# Autodesk Inventor assembly: RCR_ArmAssemblyFinal
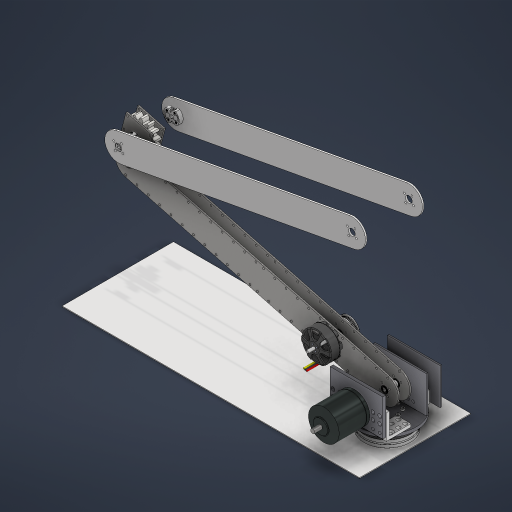
[picture p0: Inventor's stored thumbnail of the model, 512x512]
Saved by Autodesk Inventor 2024 (Build 280153000, 153)
## iProperties
Created: 2023-11-20
Part Number: RCR_ArmAssemblyFinal
Document SubType Name: Assembly
Designer: avsar
Author: avsar
## Documents named in this file (24)
- C:\Users\avsar\Documents\Inventor\RCR_Arm_Temp\ArmFinal\RCR_ArmAssemblyFinal.iam
- C:\Users\avsar\Documents\Inventor\RCR_Arm_Temp\Chassis\ChassisTop V3.ipt
- C:\Users\avsar\Documents\Inventor\RCR_Arm_Temp\COTS\Motion\Bearings\Crossed Roller Bearings\35mm Shaft Crossed Roller Bearing.ipt
- C:\Users\avsar\Documents\Inventor\RCR_Arm_Temp\ArmFinal\Turret\TurretPulley.ipt
- C:\Users\avsar\Documents\Inventor\RCR_Arm_Temp\ArmFinal\Turret\TurretBasePlate.ipt
- C:\Users\avsar\Documents\Inventor\RCR_Arm_Temp\COTS\ISO Standard Hardware\Screws\Sockethead Screws\Cap Screws\M4 x 0.7mm\(M4 x 0.7 x 30) Sockethead Cap Screw.ipt
- C:\Users\avsar\Documents\Inventor\RCR_Arm_Temp\COTS\Motion\Actuation\Motors\BLDC Motors\ODrive BLDC Motor - D6374 150KV.ipt
- C:\Users\avsar\Documents\Inventor\RCR_Arm_Temp\COTS\Motion\Actuation\Motors\BLDC Motors\ODrive Dual Shaft Motor - D5312s 330KV.ipt
- C:\Users\avsar\Documents\Inventor\RCR_Arm_Temp\ArmFinal\ArmStages\FirstStageMotorPlate.ipt
- C:\Users\avsar\Documents\Inventor\RCR_Arm_Temp\ArmFinal\ArmStages\ArmSupportPlate.ipt
- C:\Users\avsar\Documents\Inventor\RCR_Arm_Temp\ArmFinal\ArmStages\FirstStageArmBar1.ipt
- C:\Users\avsar\Documents\Inventor\RCR_Arm_Temp\COTS\goBilda\Motion\Bearings\(8mm REX ID x 14mm OD, 5mm Thickness) 1611 Series Flanged Ball Bearing.ipt
- C:\Users\avsar\Documents\Inventor\RCR_Arm_Temp\ArmFinal\ArmStages\ArmPlateSpacerFirstStage.ipt
- C:\Users\avsar\Documents\Inventor\RCR_Arm_Temp\COTS\goBilda\Motion\Collars\8mm REX-Shaft Set Screw Collar.ipt
- C:\Users\avsar\Documents\Inventor\RCR_Arm_Temp\ArmFinal\ArmStages\FirstArmStageSupportSpacer.ipt
- C:\Users\avsar\Documents\Inventor\RCR_Arm_Temp\COTS\ISO Standard Hardware\Screws\Sockethead Screws\Cap Screws\M4 x 0.7mm\(M4 x 0.7 x 8) Sockethead Cap Screw.ipt
- C:\Users\avsar\Documents\Inventor\RCR_Arm_Temp\ArmFinal\ArmStages\LongL-Bracket.ipt
- C:\Users\avsar\Documents\Inventor\RCR_Arm_Temp\ArmFinal\ArmStages\SecondArmStageMotorPulley.ipt
- C:\Users\avsar\Documents\Inventor\RCR_Arm_Temp\COTS\goBilda\Motion\Hubs\Sonic Hubs\Sonic Hub (8mm REX Bore).ipt
- C:\Users\avsar\Documents\Inventor\RCR_Arm_Temp\COTS\goBilda\Motion\Axles\(8mm Diameter, 56mm Length) 2106 Series Threaded REX Shaft with E-Clip.ipt
- C:\Users\avsar\Documents\Inventor\RCR_Arm_Temp\COTS\goBilda\Motion\Collars\Clamping Collar (8mm Rex).ipt
- C:\Users\avsar\Documents\Inventor\RCR_Arm_Temp\ArmFinal\ArmStages\SecondStageGears\ArmGears_SecondStage\Design Accelerator\Spur Gear11.ipt
- C:\Users\avsar\Documents\Inventor\RCR_Arm_Temp\ArmFinal\ArmStages\SecondStageArmBar.ipt
- C:\Users\avsar\Documents\Inventor\RCR_Arm_Temp\ArmFinal\ArmStages\ArmSupport_C-Channel.ipt
## Components (49 placed, 23 different names)
1. ChassisTop V3:1 — Mate:1, Mate:2, Mate:3
2. 35mm Shaft Crossed Roller Bearing:1 — Mate:1, Mate:2, Mate:3, Mate:4, Mate:5
3. TurretPulley:1 — Mate:4, Mate:5, Mate:6, Mate:7, Mate:8
4. (M4 x 0.7 x 30) Sockethead Cap Screw:1 — Mate:13, Mate:14
5. (M4 x 0.7 x 30) Sockethead Cap Screw:2 — Mate:11, Mate:12
6. (M4 x 0.7 x 30) Sockethead Cap Screw:3 — Mate:9, Mate:10
7. (M4 x 0.7 x 30) Sockethead Cap Screw:4 — Mate:19, Mate:20
8. (M4 x 0.7 x 30) Sockethead Cap Screw:5 — Mate:17, Mate:18
9. (M4 x 0.7 x 30) Sockethead Cap Screw:6 — Mate:15, Mate:16
10. TurretBasePlate:1 — Mate:6, Mate:7, Mate:8, Mate:9, Mate:10, Mate:11, Mate:12, Mate:13, Mate:14, Mate:15, Mate:16, Mate:17, Mate:18, Mate:19, Mate:20, Mate:21, Mate:22, Mate:23, Mate:24, Mate:77, Mate:80, Mate:119, Mate:120, Mate:121
11. (M4 x 0.7 x 30) Sockethead Cap Screw:7 — Mate:23, Mate:24
12. (M4 x 0.7 x 30) Sockethead Cap Screw:8 — Mate:21, Mate:22
13. ODrive Dual Shaft Motor - D5312s 330KV:1 — Mate:52, Mate:53, Mate:54
14. FirstStageMotorPlate:1 — Mate:36, Mate:37, Mate:38, Mate:70, Mate:71, Mate:74, Mate:75, Mate:76, Mate:78, Mate:79
15. ODrive BLDC Motor - D6374 150KV:3 — Mate:36, Mate:37, Mate:38, Mate:51
16. ArmSupportPlate:1 — Mate:123, Mate:126, Mate:127
17. ArmSupportPlate:2 — Mate:65, Mate:66, Mate:122, Mate:124, Mate:125
18. FirstStageArmBar1:1 — Mate:51, Mate:52, Mate:53, Mate:54, Mate:55, Flush:2, Mate:56, Mate:57, Mate:89, Mate:90, Mate:91, Mate:92, Mate:106
19. FirstStageArmBar1:2 — Mate:55, Flush:2, Mate:58, Mate:59, Mate:81, Mate:82, Mate:86, Mate:87, Mate:88, Mate:93, Mate:94
20. (8mm REX ID x 14mm OD, 5mm Thickness) 1611 Series Flanged Ball Bearing:1 — Mate:56, Mate:57, Mate:62
21. (8mm REX ID x 14mm OD, 5mm Thickness) 1611 Series Flanged Ball Bearing:2 — Mate:58, Mate:59, Mate:60, Mate:61, Mate:69
22. ArmPlateSpacerFirstStage:1 — Mate:60, Mate:61, Mate:63, Mate:64, Mate:68
23. 8mm REX-Shaft Set Screw Collar:1 — Mate:62, Mate:63, Mate:64
24. (8mm REX ID x 14mm OD, 5mm Thickness) 1611 Series Flanged Ball Bearing:3 — Mate:65, Mate:66, Mate:67, Mate:128
25. FirstArmStageSupportSpacer:1 — Mate:67, Mate:68, Mate:69, Mate:128
26. (M4 x 0.7 x 8) Sockethead Cap Screw:1 — Mate:70, Mate:71
27. (M4 x 0.7 x 8) Sockethead Cap Screw:2 — Mate:74, Mate:75
28. LongL-Bracket:1 — Mate:76, Mate:77, Mate:78, Mate:79, Mate:80
29. SecondArmStageMotorPulley:1 — Mate:81, Mate:82, Flush:3
30. SecondArmStageMotorPulley:2 — Mate:83, Mate:84, Mate:85, Flush:3, Mate:86, Mate:95, Mate:96
31. Sonic Hub (8mm REX Bore):1 — Mate:83, Mate:84, Mate:85
32. (8mm REX ID x 14mm OD, 5mm Thickness) 1611 Series Flanged Ball Bearing:4 — Mate:87, Mate:88
33. (8mm REX ID x 14mm OD, 5mm Thickness) 1611 Series Flanged Ball Bearing:5 — Mate:89, Mate:90, Mate:97, Mate:98
34. (8mm REX ID x 14mm OD, 5mm Thickness) 1611 Series Flanged Ball Bearing:6 — Mate:91, Mate:92, Mate:110, Mate:112, Mate:129, Mate:130
35. (8mm REX ID x 14mm OD, 5mm Thickness) 1611 Series Flanged Ball Bearing:7 — Mate:93, Mate:94, Mate:111, Mate:131, Mate:132
36. (8mm REX ID x 14mm OD, 5mm Thickness) 1611 Series Flanged Ball Bearing:8 — Mate:95, Mate:96, Mate:99
37. (8mm Diameter, 56mm Length) 2106 Series Threaded REX Shaft with E-Clip:1 — Mate:97, Mate:98, Mate:100, Mate:101, Mate:105
38. Clamping Collar (8mm Rex):1 — Mate:99, Mate:100, Mate:101
39. Spur Gear1:1 — Mate:102, Mate:103, Mate:104, Mate:105, Mate:106, Flush:4
40. Sonic Hub (8mm REX Bore):2 — Mate:102, Mate:103, Mate:104
41. Spur Gear1:2 — Mate:110, Flush:4
42. Sonic Hub (8mm REX Bore):3 — Flush:8
43. SecondStageArmBar:1 — Mate:111, Flush:5, Mate:113, Mate:114, Mate:115
44. SecondStageArmBar:2 — Mate:112, Flush:5, Mate:116, Mate:117, Mate:118
45. Sonic Hub (8mm REX Bore):4 — Mate:113, Mate:114, Mate:115, Flush:6, Flush:7, Flush:8
46. Sonic Hub (8mm REX Bore):5 — Mate:116, Mate:117, Mate:118, Mate:133
47. ArmSupport_C-Channel:1 — Mate:119, Mate:120, Mate:121, Mate:122, Mate:123, Mate:124, Mate:125, Mate:126, Mate:127
48. Clamping Collar (8mm Rex):2 — Mate:129, Mate:130, Flush:6
49. Clamping Collar (8mm Rex):3 — Mate:131, Mate:132, Flush:7, Mate:133
## Relationships (115: Mate 108, Flush 7)
- Mate:1: ChassisTop V3:1 ↔ 35mm Shaft Crossed Roller Bearing:1
- Mate:2: ChassisTop V3:1 ↔ 35mm Shaft Crossed Roller Bearing:1
- Mate:3: ChassisTop V3:1 ↔ 35mm Shaft Crossed Roller Bearing:1
- Mate:4: 35mm Shaft Crossed Roller Bearing:1 ↔ TurretPulley:1
- Mate:5: 35mm Shaft Crossed Roller Bearing:1 ↔ TurretPulley:1
- Mate:6: TurretPulley:1 ↔ TurretBasePlate:1
- Mate:7: TurretPulley:1 ↔ TurretBasePlate:1
- Mate:8: TurretPulley:1 ↔ TurretBasePlate:1
- Mate:9: (M4 x 0.7 x 30) Sockethead Cap Screw:3 ↔ TurretBasePlate:1
- Mate:10: (M4 x 0.7 x 30) Sockethead Cap Screw:3 ↔ TurretBasePlate:1
- Mate:11: (M4 x 0.7 x 30) Sockethead Cap Screw:2 ↔ TurretBasePlate:1
- Mate:12: (M4 x 0.7 x 30) Sockethead Cap Screw:2 ↔ TurretBasePlate:1
- Mate:13: (M4 x 0.7 x 30) Sockethead Cap Screw:1 ↔ TurretBasePlate:1
- Mate:14: (M4 x 0.7 x 30) Sockethead Cap Screw:1 ↔ TurretBasePlate:1
- Mate:15: (M4 x 0.7 x 30) Sockethead Cap Screw:6 ↔ TurretBasePlate:1
- Mate:16: (M4 x 0.7 x 30) Sockethead Cap Screw:6 ↔ TurretBasePlate:1
- Mate:17: (M4 x 0.7 x 30) Sockethead Cap Screw:5 ↔ TurretBasePlate:1
- Mate:18: (M4 x 0.7 x 30) Sockethead Cap Screw:5 ↔ TurretBasePlate:1
- Mate:19: (M4 x 0.7 x 30) Sockethead Cap Screw:4 ↔ TurretBasePlate:1
- Mate:20: (M4 x 0.7 x 30) Sockethead Cap Screw:4 ↔ TurretBasePlate:1
- Mate:21: TurretBasePlate:1 ↔ (M4 x 0.7 x 30) Sockethead Cap Screw:8
- Mate:22: TurretBasePlate:1 ↔ (M4 x 0.7 x 30) Sockethead Cap Screw:8
- Mate:23: TurretBasePlate:1 ↔ (M4 x 0.7 x 30) Sockethead Cap Screw:7
- Mate:24: TurretBasePlate:1 ↔ (M4 x 0.7 x 30) Sockethead Cap Screw:7
- Mate:36: FirstStageMotorPlate:1 ↔ ODrive BLDC Motor - D6374 150KV:3
- Mate:37: FirstStageMotorPlate:1 ↔ ODrive BLDC Motor - D6374 150KV:3
- Mate:38: FirstStageMotorPlate:1 ↔ ODrive BLDC Motor - D6374 150KV:3
- Mate:51: ODrive BLDC Motor - D6374 150KV:3 ↔ FirstStageArmBar1:1
- Mate:52: ODrive Dual Shaft Motor - D5312s 330KV:1 ↔ FirstStageArmBar1:1
- Mate:53: ODrive Dual Shaft Motor - D5312s 330KV:1 ↔ FirstStageArmBar1:1
- Mate:54: ODrive Dual Shaft Motor - D5312s 330KV:1 ↔ FirstStageArmBar1:1
- Mate:55: FirstStageArmBar1:1 ↔ FirstStageArmBar1:2
- Flush:2: FirstStageArmBar1:1 ↔ FirstStageArmBar1:2
- Mate:56: FirstStageArmBar1:1 ↔ (8mm REX ID x 14mm OD, 5mm Thickness) 1611 Series Flanged Ball Bearing:1
- Mate:57: FirstStageArmBar1:1 ↔ (8mm REX ID x 14mm OD, 5mm Thickness) 1611 Series Flanged Ball Bearing:1
- Mate:58: FirstStageArmBar1:2 ↔ (8mm REX ID x 14mm OD, 5mm Thickness) 1611 Series Flanged Ball Bearing:2
- Mate:59: FirstStageArmBar1:2 ↔ (8mm REX ID x 14mm OD, 5mm Thickness) 1611 Series Flanged Ball Bearing:2
- Mate:60: (8mm REX ID x 14mm OD, 5mm Thickness) 1611 Series Flanged Ball Bearing:2 ↔ ArmPlateSpacerFirstStage:1
- Mate:61: (8mm REX ID x 14mm OD, 5mm Thickness) 1611 Series Flanged Ball Bearing:2 ↔ ArmPlateSpacerFirstStage:1
- Mate:62: (8mm REX ID x 14mm OD, 5mm Thickness) 1611 Series Flanged Ball Bearing:1 ↔ 8mm REX-Shaft Set Screw Collar:1
- Mate:63: ArmPlateSpacerFirstStage:1 ↔ 8mm REX-Shaft Set Screw Collar:1
- Mate:64: ArmPlateSpacerFirstStage:1 ↔ 8mm REX-Shaft Set Screw Collar:1
- Mate:65: ArmSupportPlate:2 ↔ (8mm REX ID x 14mm OD, 5mm Thickness) 1611 Series Flanged Ball Bearing:3
- Mate:66: ArmSupportPlate:2 ↔ (8mm REX ID x 14mm OD, 5mm Thickness) 1611 Series Flanged Ball Bearing:3
- Mate:67: (8mm REX ID x 14mm OD, 5mm Thickness) 1611 Series Flanged Ball Bearing:3 ↔ FirstArmStageSupportSpacer:1
- Mate:68: ArmPlateSpacerFirstStage:1 ↔ FirstArmStageSupportSpacer:1
- Mate:69: (8mm REX ID x 14mm OD, 5mm Thickness) 1611 Series Flanged Ball Bearing:2 ↔ FirstArmStageSupportSpacer:1
- Mate:70: FirstStageMotorPlate:1 ↔ (M4 x 0.7 x 8) Sockethead Cap Screw:1
- Mate:71: FirstStageMotorPlate:1 ↔ (M4 x 0.7 x 8) Sockethead Cap Screw:1
- Mate:74: FirstStageMotorPlate:1 ↔ (M4 x 0.7 x 8) Sockethead Cap Screw:2
- Mate:75: FirstStageMotorPlate:1 ↔ (M4 x 0.7 x 8) Sockethead Cap Screw:2
- Mate:76: FirstStageMotorPlate:1 ↔ LongL-Bracket:1
- Mate:77: TurretBasePlate:1 ↔ LongL-Bracket:1
- Mate:78: FirstStageMotorPlate:1 ↔ LongL-Bracket:1
- Mate:79: FirstStageMotorPlate:1 ↔ LongL-Bracket:1
- Mate:80: TurretBasePlate:1 ↔ LongL-Bracket:1
- Mate:81 (4 mm): FirstStageArmBar1:2 ↔ SecondArmStageMotorPulley:1
- Mate:82: FirstStageArmBar1:2 ↔ SecondArmStageMotorPulley:1
- Mate:83: SecondArmStageMotorPulley:2 ↔ Sonic Hub (8mm REX Bore):1
- Mate:84: SecondArmStageMotorPulley:2 ↔ Sonic Hub (8mm REX Bore):1
- Mate:85: SecondArmStageMotorPulley:2 ↔ Sonic Hub (8mm REX Bore):1
- Flush:3: SecondArmStageMotorPulley:1 ↔ SecondArmStageMotorPulley:2
- Mate:86: FirstStageArmBar1:2 ↔ SecondArmStageMotorPulley:2
- Mate:87: FirstStageArmBar1:2 ↔ (8mm REX ID x 14mm OD, 5mm Thickness) 1611 Series Flanged Ball Bearing:4
- Mate:88: FirstStageArmBar1:2 ↔ (8mm REX ID x 14mm OD, 5mm Thickness) 1611 Series Flanged Ball Bearing:4
- Mate:89: FirstStageArmBar1:1 ↔ (8mm REX ID x 14mm OD, 5mm Thickness) 1611 Series Flanged Ball Bearing:5
- Mate:90: FirstStageArmBar1:1 ↔ (8mm REX ID x 14mm OD, 5mm Thickness) 1611 Series Flanged Ball Bearing:5
- Mate:91: FirstStageArmBar1:1 ↔ (8mm REX ID x 14mm OD, 5mm Thickness) 1611 Series Flanged Ball Bearing:6
- Mate:92: FirstStageArmBar1:1 ↔ (8mm REX ID x 14mm OD, 5mm Thickness) 1611 Series Flanged Ball Bearing:6
- Mate:93: FirstStageArmBar1:2 ↔ (8mm REX ID x 14mm OD, 5mm Thickness) 1611 Series Flanged Ball Bearing:7
- Mate:94: FirstStageArmBar1:2 ↔ (8mm REX ID x 14mm OD, 5mm Thickness) 1611 Series Flanged Ball Bearing:7
- Mate:95: SecondArmStageMotorPulley:2 ↔ (8mm REX ID x 14mm OD, 5mm Thickness) 1611 Series Flanged Ball Bearing:8
- Mate:96: SecondArmStageMotorPulley:2 ↔ (8mm REX ID x 14mm OD, 5mm Thickness) 1611 Series Flanged Ball Bearing:8
- Mate:97: (8mm REX ID x 14mm OD, 5mm Thickness) 1611 Series Flanged Ball Bearing:5 ↔ (8mm Diameter, 56mm Length) 2106 Series Threaded REX Shaft with E-Clip:1
- Mate:98: (8mm REX ID x 14mm OD, 5mm Thickness) 1611 Series Flanged Ball Bearing:5 ↔ (8mm Diameter, 56mm Length) 2106 Series Threaded REX Shaft with E-Clip:1
- Mate:99: (8mm REX ID x 14mm OD, 5mm Thickness) 1611 Series Flanged Ball Bearing:8 ↔ Clamping Collar (8mm Rex):1
- Mate:100: (8mm Diameter, 56mm Length) 2106 Series Threaded REX Shaft with E-Clip:1 ↔ Clamping Collar (8mm Rex):1
- Mate:101: (8mm Diameter, 56mm Length) 2106 Series Threaded REX Shaft with E-Clip:1 ↔ Clamping Collar (8mm Rex):1
- Mate:102: Spur Gear1:1 ↔ Sonic Hub (8mm REX Bore):2
- Mate:103: Spur Gear1:1 ↔ Sonic Hub (8mm REX Bore):2
- Mate:104: Spur Gear1:1 ↔ Sonic Hub (8mm REX Bore):2
- Mate:105: (8mm Diameter, 56mm Length) 2106 Series Threaded REX Shaft with E-Clip:1 ↔ Spur Gear1:1
- Mate:106 (4 mm): FirstStageArmBar1:1 ↔ Spur Gear1:1
- [Mate]: Spur Gear1:2 ↔ Sonic Hub (8mm REX Bore):3
- [Mate]: Spur Gear1:2 ↔ Sonic Hub (8mm REX Bore):3
- [Mate]: Spur Gear1:2 ↔ Sonic Hub (8mm REX Bore):3
- Mate:110: (8mm REX ID x 14mm OD, 5mm Thickness) 1611 Series Flanged Ball Bearing:6 ↔ Spur Gear1:2
- Flush:4: Spur Gear1:1 ↔ Spur Gear1:2
- Mate:111: (8mm REX ID x 14mm OD, 5mm Thickness) 1611 Series Flanged Ball Bearing:7 ↔ SecondStageArmBar:1
- Mate:112: (8mm REX ID x 14mm OD, 5mm Thickness) 1611 Series Flanged Ball Bearing:6 ↔ SecondStageArmBar:2
- Flush:5: SecondStageArmBar:1 ↔ SecondStageArmBar:2
- Mate:113: SecondStageArmBar:1 ↔ Sonic Hub (8mm REX Bore):4
- Mate:114: SecondStageArmBar:1 ↔ Sonic Hub (8mm REX Bore):4
- Mate:115: SecondStageArmBar:1 ↔ Sonic Hub (8mm REX Bore):4
- Mate:116: SecondStageArmBar:2 ↔ Sonic Hub (8mm REX Bore):5
- Mate:117: SecondStageArmBar:2 ↔ Sonic Hub (8mm REX Bore):5
- Mate:118: SecondStageArmBar:2 ↔ Sonic Hub (8mm REX Bore):5
- Mate:119: TurretBasePlate:1 ↔ ArmSupport_C-Channel:1
- Mate:120: TurretBasePlate:1 ↔ ArmSupport_C-Channel:1
- Mate:121: TurretBasePlate:1 ↔ ArmSupport_C-Channel:1
- Mate:122: ArmSupportPlate:2 ↔ ArmSupport_C-Channel:1
- Mate:123: ArmSupportPlate:1 ↔ ArmSupport_C-Channel:1
- Mate:124: ArmSupportPlate:2 ↔ ArmSupport_C-Channel:1
- Mate:125: ArmSupportPlate:2 ↔ ArmSupport_C-Channel:1
- Mate:126: ArmSupportPlate:1 ↔ ArmSupport_C-Channel:1
- Mate:127: ArmSupportPlate:1 ↔ ArmSupport_C-Channel:1
- Mate:128: (8mm REX ID x 14mm OD, 5mm Thickness) 1611 Series Flanged Ball Bearing:3 ↔ FirstArmStageSupportSpacer:1
- Mate:129: (8mm REX ID x 14mm OD, 5mm Thickness) 1611 Series Flanged Ball Bearing:6 ↔ Clamping Collar (8mm Rex):2
- Mate:130: (8mm REX ID x 14mm OD, 5mm Thickness) 1611 Series Flanged Ball Bearing:6 ↔ Clamping Collar (8mm Rex):2
- Flush:6: Sonic Hub (8mm REX Bore):4 ↔ Clamping Collar (8mm Rex):2
- Mate:131: (8mm REX ID x 14mm OD, 5mm Thickness) 1611 Series Flanged Ball Bearing:7 ↔ Clamping Collar (8mm Rex):3
- Mate:132: (8mm REX ID x 14mm OD, 5mm Thickness) 1611 Series Flanged Ball Bearing:7 ↔ Clamping Collar (8mm Rex):3
- Flush:7: Sonic Hub (8mm REX Bore):4 ↔ Clamping Collar (8mm Rex):3
- Mate:133 (36 mm): Sonic Hub (8mm REX Bore):5 ↔ Clamping Collar (8mm Rex):3
- Flush:8: Sonic Hub (8mm REX Bore):3 ↔ Sonic Hub (8mm REX Bore):4
## Named parameters: d147_d142 = 0 mm, d148_d143 = 0 mm, d149_d144 = 0 mm
